# Autodesk Inventor assembly: 新款V5 2号螺丝螺帽套
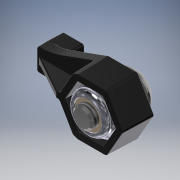
[picture p0: Inventor's stored thumbnail of the model, 180x180]
Saved by Autodesk Inventor 2019.3 (Build 233278000, 278)
## iProperties
Created: 2019-03-29
Part Number: 新款V5 2号螺丝螺帽套
Material: 常规
Document SubType Name: Assembly
Designer: aresp
Author: aresp
## Documents named in this file (4)
- D:\cad\零件库\新款V5 2号螺丝螺帽套.iam
- D:\cad\零件库\螺丝螺帽\Nut 8-32 Nylock.ipt
- D:\cad\零件库\螺丝螺帽\Screw 8-32 x 0.375'' - Black.ipt
- D:\cad\零件库\垫片轴套大白等\1-Post_Hex_Nut_Retainer_276-6482.ipt
## Components (3 placed, 3 different names)
1. Nut 8-32 Nylock:1 — 配合:1, 配合:2, 配合:4
2. Screw 8-32 x 0.375'' - Black:1 — 配合:3, 配合:4
3. 1-Post_Hex_Nut_Retainer_276-6482:1 — 配合:1, 配合:2, 配合:3
## Relationships (4: Mate 4)
- 配合:1 [Mate]: Nut 8-32 Nylock:1 ↔ 1-Post_Hex_Nut_Retainer_276-6482:1
- 配合:2 [Mate]: Nut 8-32 Nylock:1 ↔ 1-Post_Hex_Nut_Retainer_276-6482:1
- 配合:3 [Mate] (1.6 mm): Screw 8-32 x 0.375'' - Black:1 ↔ 1-Post_Hex_Nut_Retainer_276-6482:1
- 配合:4 [Mate]: Nut 8-32 Nylock:1 ↔ Screw 8-32 x 0.375'' - Black:1
